# Autodesk Inventor assembly: EL2-A-100
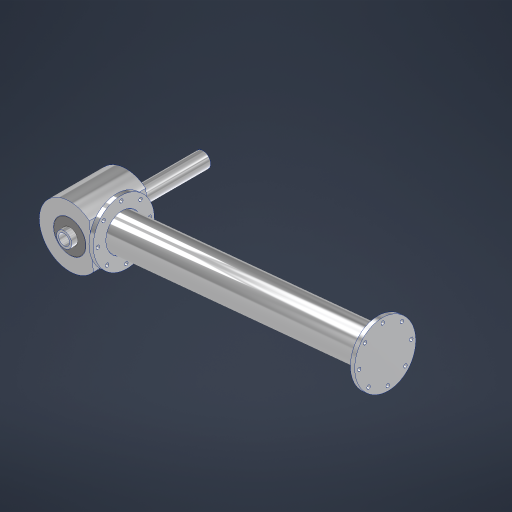
[picture p0: Inventor's stored thumbnail of the model, 512x512]
Saved by Autodesk Inventor 2023.4 (Build 274418000, 418)
## iProperties
Created: 2025-01-11
Part Number: EL2-A-100
Document SubType Name: Assembly
Designer: brand
Mass: 2250.36 g
Surface Area: 2618 cm^2
Volume: 766.484 cm^3
Density: 2.93596 g/cm^3
Author: brand
## Documents named in this file (6)
- C:\Users\brand\OneDrive\Documents\GitHub\robotics 23\2025-ReefScape---CAD\Elevator\EL2\EL2-A-100.iam
- C:\Users\brand\OneDrive\Documents\GitHub\robotics 23\2025-ReefScape---CAD\Elevator\EL2\EL2-A-002.ipt
- C:\Users\brand\OneDrive\Documents\GitHub\robotics 23\2025-ReefScape---CAD\Elevator\EL2\EL2-A-003.ipt
- C:\Users\brand\OneDrive\Documents\GitHub\robotics 23\2025-ReefScape---CAD\COMMON PARTS\BEARINGS\0_875_ID_x_1_875_OD_X_0_500_Radial_Bearing_EE11S-2RS.ipt
- C:\Users\brand\OneDrive\Documents\GitHub\robotics 23\2025-ReefScape---CAD\Elevator\EL2\EL2-A-004.ipt
- C:\Users\brand\OneDrive\Documents\GitHub\robotics 23\2025-ReefScape---CAD\Elevator\EL2\EL2-A-005.ipt
## Components (7 placed, 5 different names)
1. EL2-A-005:1 — Mate:1
2. EL2-A-002:1 — Insert:1, Flush:1, Insert:2, Flush:2
3. EL2-A-003:1 — Insert:1, Flush:1, Insert:5, Insert:6
4. EL2-A-003:2 — Insert:2, Flush:2
5. 0_875_ID_x_1_875_OD_X_0_500_Radial_Bearing_EE11S-2RS:1 — Insert:4
6. 0_875_ID_x_1_875_OD_X_0_500_Radial_Bearing_EE11S-2RS:2 — Insert:3, Mate:1
7. EL2-A-004:1 — Insert:3, Insert:4, Insert:5, Insert:6
## Relationships (9: Insert 6, Flush 2, Mate 1)
- Insert:1: EL2-A-002:1 ↔ EL2-A-003:1
- Flush:1: EL2-A-002:1 ↔ EL2-A-003:1
- Insert:2: EL2-A-002:1 ↔ EL2-A-003:2
- Flush:2: EL2-A-002:1 ↔ EL2-A-003:2
- Insert:3: 0_875_ID_x_1_875_OD_X_0_500_Radial_Bearing_EE11S-2RS:2 ↔ EL2-A-004:1
- Insert:4: 0_875_ID_x_1_875_OD_X_0_500_Radial_Bearing_EE11S-2RS:1 ↔ EL2-A-004:1
- Mate:1: EL2-A-005:1 ↔ 0_875_ID_x_1_875_OD_X_0_500_Radial_Bearing_EE11S-2RS:2
- Insert:5: EL2-A-003:1 ↔ EL2-A-004:1
- Insert:6: EL2-A-003:1 ↔ EL2-A-004:1
